# Autodesk Inventor assembly: Power Expander
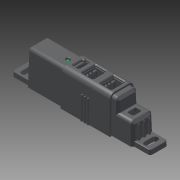
[picture p0: Inventor's stored thumbnail of the model, 180x180]
Saved by Autodesk Inventor 2014 SP1 (Build 180222100, 222)
## iProperties
Created: 2011-03-21
Part Number: Power Expander
Document SubType Name: Assembly
Designer: Jordan
Translation Standard: STEP AP203
FileName: VEX-POWER-EXPANDER.STEP
PreProcessor: SolidWorks 2010
PostProcessor: Build: 239, Release: 2011 RTM - Date: Wed 02/17/2010
Sent Units: inch
Uncertainty: 1e-05
Author: Jordan
## Documents named in this file (5)
- C:\Users\Ryan\Desktop\pack and go\Workspaces\Workspace\lib\Super Sonic Sparks VEX CAD Library\Other Parts\Power Expander.iam
- C:\Users\Ryan\Desktop\pack and go\Workspaces\Workspace\lib\Super Sonic Sparks VEX CAD Library\Other Parts\Power Expander-Parts\LED.ipt
- C:\Users\Ryan\Desktop\pack and go\Workspaces\Workspace\lib\Super Sonic Sparks VEX CAD Library\Other Parts\Power Expander-Parts\Bottom Case.ipt
- C:\Users\Ryan\Desktop\pack and go\Workspaces\Workspace\lib\Super Sonic Sparks VEX CAD Library\Other Parts\Power Expander-Parts\Lock Slide.ipt
- C:\Users\Ryan\Desktop\pack and go\Workspaces\Workspace\lib\Super Sonic Sparks VEX CAD Library\Other Parts\Power Expander-Parts\Top Case.ipt
## Components (4 placed, 4 different names)
1. LED:1
2. Bottom Case:1 — Flush:2, Flush:3, Flush:4
3. Lock Slide:1
4. Top Case:1 — Flush:1
## Relationships (6: Flush 4, Mate 2)
- Flush:1 (-0.762 mm): Top Case:1
- Flush:2 (2.1717 mm): Bottom Case:1
- Flush:3 (2.1717 mm): Bottom Case:1
- Flush:4 (2.1717 mm): Bottom Case:1
- Mate:1
- Mate:2
